# Autodesk Inventor assembly: motormounted
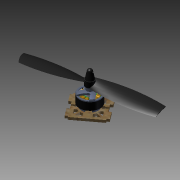
[picture p0: Inventor's stored thumbnail of the model, 180x180]
Saved by Autodesk Inventor 2012 (Build 160160000, 160)
## iProperties
Created: 2014-07-10
Part Number: motormounted
Document SubType Name: Assembly
Designer: Anon
Author: Anon
## Documents named in this file (4)
- D:\Dropbox\Courses\GP\Inventor\dronestructure\motor\motormounted.iam
- D:\Dropbox\Courses\GP\Inventor\dronestructure\motor\motorassembly.iam
- D:\Dropbox\Courses\GP\Inventor\dronestructure\MotorSupport.ipt
- C:\Users\Anon\Documents\Inventor\Content Center Files\R2012\en-US\JIS B 1176\JIS B 1176 - M3 x 6.ipt
## Components (6 placed, 3 different names)
1. motorassembly:1 [sub-assembly] — Mate:1, Mate:2, Mate:3
2. MotorSupport:1 — Mate:1, Mate:2, Mate:3, Mate:4, Mate:5, Mate:6, Mate:7, Mate:8, Mate:9, Mate:10, Mate:11
3. JIS B 1176 - Metric M3 x 6:1 — Mate:6, Mate:7
4. JIS B 1176 - Metric M3 x 6:2 — Mate:4, Mate:5
5. JIS B 1176 - Metric M3 x 6:3 — Mate:8, Mate:9
6. JIS B 1176 - Metric M3 x 6:4 — Mate:10, Mate:11
## Relationships (11: Mate 11)
- Mate:1: motorassembly:1 ↔ MotorSupport:1
- Mate:2: motorassembly:1 ↔ MotorSupport:1
- Mate:3: motorassembly:1 ↔ MotorSupport:1
- Mate:4: MotorSupport:1 ↔ JIS B 1176 - Metric M3 x 6:2
- Mate:5: MotorSupport:1 ↔ JIS B 1176 - Metric M3 x 6:2
- Mate:6: MotorSupport:1 ↔ JIS B 1176 - Metric M3 x 6:1
- Mate:7: MotorSupport:1 ↔ JIS B 1176 - Metric M3 x 6:1
- Mate:8: MotorSupport:1 ↔ JIS B 1176 - Metric M3 x 6:3
- Mate:9: MotorSupport:1 ↔ JIS B 1176 - Metric M3 x 6:3
- Mate:10: MotorSupport:1 ↔ JIS B 1176 - Metric M3 x 6:4
- Mate:11: MotorSupport:1 ↔ JIS B 1176 - Metric M3 x 6:4
